# Autodesk Inventor assembly: axis3
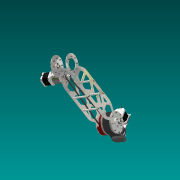
[picture p0: Inventor's stored thumbnail of the model, 180x180]
Saved by Autodesk Inventor 2020 (Build 240168000, 168)
## iProperties
Created: 2020-05-24
Part Number: axis3
Document SubType Name: Assembly
Designer: Svend
Author: Svend
## Documents named in this file (27)
- D:\github_gedeeld\BeerMinder\3D-model\axis3\axis3.iam
- D:\github_gedeeld\BeerMinder\3D-model\subAssembly\Nema17MetGearbox.iam
- D:\github_gedeeld\BeerMinder\3D-model\pulleys\GT2 Timing Pulley 20T - 8mm as.ipt
- D:\github_gedeeld\BeerMinder\3D-model\pulleys\Tandriem20naar60T-696mm.ipt
- D:\github_gedeeld\BeerMinder\3D-model\Base (Axis 1)\spiebaanBevestiging.ipt
- D:\github_gedeeld\BeerMinder\3D-model\pulleys\GT2 Timing Pulley 60T - 8mm as.ipt
- D:\github_gedeeld\BeerMinder\3D-model\bearings\Ball Bearing 608ZZ.ipt
- D:\github_gedeeld\BeerMinder\3D-model\Base (Axis 1)\asArm2.ipt
- D:\github_gedeeld\BeerMinder\3D-model\Base (Axis 1)\arm1v2.ipt
- D:\github_gedeeld\BeerMinder\3D-model\Base (Axis 1)\60mmspacer.ipt
- D:\github_gedeeld\BeerMinder\3D-model\Base (Axis 1)\60mmspacerDicht.ipt
- D:\github_gedeeld\BeerMinder\3D-model\bearings\stelring - 8mm.ipt
- D:\github_gedeeld\BeerMinder\3D-model\axis4\spacerVoorLager.ipt
- D:\github_gedeeld\BeerMinder\3D-model\boutjesEnMoertjes\ISO 4762 - M3 x 10ISO.ipt
- D:\github_gedeeld\BeerMinder\3D-model\boutjesEnMoertjes\ISO 7089 - 3 - 140 HV(1).ipt
- D:\github_gedeeld\BeerMinder\3D-model\boutjesEnMoertjes\ISO 10642 - M3x12.ipt
- D:\github_gedeeld\BeerMinder\3D-model\boutjesEnMoertjes\ISO 4035 - M3 - ISO.ipt
- D:\github_gedeeld\BeerMinder\3D-model\Base (Axis 1)\spiebaanplaatKlein.ipt
- D:\github_gedeeld\BeerMinder\3D-model\boutjesEnMoertjes\ISO 7380-1 - M4 x 16.ipt
- D:\github_gedeeld\BeerMinder\3D-model\Base (Axis 1)\arm1 tweede kant.ipt
- D:\github_gedeeld\BeerMinder\3D-model\axis4\axis4.iam
- D:\github_gedeeld\BeerMinder\3D-model\boutjesEnMoertjes\ISO 7380-1 - M3 x 8.ipt
- C:\Users\stefa\Documents\Inventor\Content Center Files\R2020\en-US\ISO 7089\ISO 7089 - 3 - 140 HV(1).ipt
- D:\github_gedeeld\BeerMinder\3D-model\axis3\asjes.ipt
- C:\Users\stefa\Documents\Inventor\Content Center Files\R2020\en-US\ISO 7089\ISO 7089 - 4 - 140 HV(1).ipt
- C:\Users\stefa\Documents\Inventor\Content Center Files\R2020\en-US\ISO 4762(2)\ISO 4762 - M4 x 12ISO.ipt
- D:\github_gedeeld\BeerMinder\3D-model\boutjesEnMoertjes\ISO 4762 - M3 x 30ISO.ipt
## Components (122 placed, 25 different names)
1. Nema17MetGearbox:1 [sub-assembly] — Mate:9, Mate:33, Mate:34, Mate:35, Mate:41
2. GT2 Timing Pulley 20T - 8mm as:1 — Mate:9, Mate:91, Mate:92
3. Tandriem20naar60T-696mm:1 — Mate:91, Mate:92
4. spiebaanBevestiging:1 — Flush:4
5. GT2 Timing Pulley 60T - 8mm as:1
6. Ball Bearing 608ZZ:1
7. asArm2:1 — Mate:89, Mate:94, Mate:98, Mate:100
8. arm1v2:1 — Mate:22, Mate:23, Mate:36, Mate:37, Mate:38, Mate:39, Mate:40, Mate:43, Mate:45, Mate:59, Insert:3, Insert:4, Insert:5, Insert:6, Insert:7, Insert:8, Insert:9, Insert:10, Mate:69, Mate:76, Insert:42, Insert:43, Insert:44, Insert:45, Insert:46, Insert:47, Insert:48, Insert:49, Mate:95, Mate:97, Mate:109, Mate:110, Insert:86, Insert:87, Insert:89, Insert:90, Insert:109, Insert:128, Mate:117, Mate:118, Mate:119
9. 60mmspacer:1
10. 60mmspacerDicht:1 — Mate:47, Mate:49, Mate:51, Mate:53, Mate:103, Mate:104
11. stelring - 8mm:1 — Mate:102
12. spacerVoorLager:1 — Mate:22, Mate:23, Mate:59, Mate:101
13. spiebaanplaatKlein:1 — Mate:69, Flush:4, Mate:70, Mate:71, Mate:72, Mate:73, Mate:74, Mate:75, Mate:76
14. 60mmspacerDicht:2 — Mate:85, Mate:86, Mate:88, Mate:90, Mate:100, Insert:72, Insert:73, Insert:74, Insert:75
15. 60mmspacer:2 — Mate:85, Mate:86, Mate:87, Mate:98, Mate:99
16. Ball Bearing 608ZZ:2 — Mate:87, Mate:88
17. stelring - 8mm:2 — Mate:89, Mate:90
18. arm1 tweede kant:1 — Mate:94, Mate:95, Mate:97, Mate:99, Insert:50, Insert:51, Insert:52, Insert:53, Insert:54, Insert:55, Insert:56, Insert:57, Insert:58, Insert:59, Insert:60, Insert:61, Insert:62, Insert:63, Insert:64, Insert:65, Mate:112, Insert:81, Insert:82, Insert:83, Insert:85, Insert:130
19. axis4:1 [sub-assembly] — Mate:101, Mate:102
20. asjes:1 — Mate:112, Mate:113
21. asjes:3 — Mate:115, Mate:117
22. asjes:4 — Mate:114, Mate:119
23. asjes:5 — Mate:116, Mate:118
24. ISO 4762 M3 x 10:12 — Insert:136
25. ISO 4762 M3 x 10:11 — Insert:135
26. ISO 4762 M3 x 10:10 — Insert:134
27. ISO 4762 M3 x 10:9 — Insert:133
28. ISO 4762 M3 x 10:8 — Insert:132
29. ISO 4762 M3 x 10:7 — Insert:131
30. ISO 4762 M3 x 10:6 — Insert:130
31. ISO 4762 M3 x 30:25 — Insert:129
32. ISO 4762 M3 x 30:24 — Insert:128
33. ISO 4762 M3 x 30:23 — Insert:127
34. ISO 4762 M3 x 30:5 — Insert:109
35. ISO 4762 M3 x 30:4 — Insert:108
36. ISO 4762 M3 x 30:3 — Insert:107
37. ISO 4762 M3 x 30:2 — Insert:106
38. ISO 4762 M3 x 30:1 — Insert:105
39. ISO 4762 M3 x 10:5 — Insert:104
40. ISO 7089 4:11 — Insert:90, Insert:99
41. ISO 7089 4:10 — Insert:89, Insert:101
42. ISO 7089 4:8 — Insert:87, Insert:100
43. ISO 7089 4:7 — Insert:86, Insert:98
44. ISO 7089 4:6 — Insert:85, Insert:95
45. ISO 7089 4:4 — Insert:83, Insert:93
46. ISO 7089 4:3 — Insert:82, Insert:94
47. ISO 7089 4:2 — Insert:81, Insert:96
48. ISO 4762 M4 x 12:10 — Insert:101
49. ISO 4762 M4 x 12:9 — Insert:100
50. ISO 4762 M4 x 12:8 — Insert:99
51. ISO 4762 M4 x 12:7 — Insert:98
52. ISO 4762 M4 x 12:5 — Insert:96, Mate:114
53. ISO 4762 M4 x 12:4 — Insert:95, Mate:115
54. ISO 4762 M4 x 12:3 — Insert:94, Mate:116
55. ISO 4762 M4 x 12:2 — Insert:93, Mate:113
56. ISO 4035 M3:8 — Insert:79, Mate:120
57. ISO 4035 M3:7 — Insert:78, Mate:123
58. ISO 4035 M3:6 — Insert:77, Mate:121
59. ISO 4035 M3:5 — Insert:76, Mate:122
60. ISO 10642 M3x12:10 — Mate:110
61. ISO 10642 M3x12:9 — Mate:109
62. ISO 10642 M3x12:8 — Mate:123
63. ISO 10642 M3x12:7 — Mate:121
64. ISO 10642 M3x12:6 — Mate:122
65. ISO 10642 M3x12:5 — Mate:120
66. ISO 7089 3:12 — Insert:75, Insert:77
67. ISO 7089 3:11 — Insert:74, Insert:78
68. ISO 7089 3:10 — Insert:73, Insert:76
69. ISO 7089 3:9 — Insert:72, Insert:79
70. ISO 7089 3:20 — Insert:65, Insert:136
71. ISO 7089 3:19 — Insert:64, Insert:134
72. ISO 7089 3:18 — Insert:63, Insert:132
73. ISO 7089 3:17 — Insert:62
74. ISO 7089 3:16 — Insert:61, Insert:131
75. ISO 7089 3:15 — Insert:60, Insert:133
76. ISO 7089 3:14 — Insert:59, Insert:135
77. ISO 7089 3:13 — Insert:58, Insert:104
78. ISO 7380-1 M3 x 8:24 — Insert:57
79. ISO 7380-1 M3 x 8:17 — Insert:56
80. ISO 7380-1 M3 x 8:18 — Insert:55
81. ISO 7380-1 M3 x 8:19 — Insert:54
82. ISO 7380-1 M3 x 8:20 — Insert:53
83. ISO 7380-1 M3 x 8:21 — Insert:52
84. ISO 7380-1 M3 x 8:22 — Insert:51
85. ISO 7380-1 M3 x 8:23 — Insert:50
86. ISO 7380-1 M3 x 8:9 — Insert:42
87. ISO 7380-1 M3 x 8:10 — Insert:43
88. ISO 7380-1 M3 x 8:11 — Insert:44
89. ISO 7380-1 M3 x 8:12 — Insert:45
90. ISO 7380-1 M3 x 8:13 — Insert:46
91. ISO 7380-1 M3 x 8:14 — Insert:47
92. ISO 7380-1 M3 x 8:15 — Insert:48
93. ISO 7380-1 M3 x 8:16 — Insert:49
94. ISO 7380-1 M4 x 16:1 — Mate:70, Mate:71
95. ISO 7380-1 M4 x 16:3 — Mate:72, Mate:73
96. ISO 7380-1 M4 x 16:2 — Mate:74, Mate:75
97. ISO 4762 M3 x 10:1 — Mate:29, Mate:30, Mate:34
98. ISO 4762 M3 x 10:2 — Mate:25, Mate:26, Mate:35
99. ISO 4762 M3 x 10:3 — Mate:27, Mate:28, Mate:41
100. ISO 4762 M3 x 10:4 — Mate:31, Mate:32, Mate:33
101. ISO 7089 3:1 — Mate:25, Mate:26, Mate:36
102. ISO 7089 3:2 — Mate:27, Mate:28, Mate:37, Mate:38
103. ISO 7089 3:3 — Mate:29, Mate:30, Mate:39
104. ISO 7089 3:4 — Mate:31, Mate:32, Mate:40
105. ISO 10642 M3x12:2 — Mate:43, Mate:46, Mate:54
106. ISO 10642 M3x12:4 — Mate:45, Mate:52, Mate:56
107. ISO 7089 3:5 — Mate:46, Mate:47, Mate:55
108. ISO 7089 3:6 — Mate:49, Insert:1
109. ISO 7089 3:7 — Mate:51, Insert:2
110. ISO 7089 3:8 — Mate:52, Mate:53, Mate:57
111. ISO 4035 M3:1 — Mate:54, Mate:55
112. ISO 4035 M3:2 — Mate:56, Mate:57
113. ISO 4035 M3:3 — Insert:1, Mate:104
114. ISO 4035 M3:4 — Insert:2, Mate:103
115. ISO 7089 3:27 — Insert:3
116. ISO 7089 3:28 — Insert:4, Insert:107
117. ISO 7089 3:29 — Insert:5, Insert:105
118. ISO 7089 3:30 — Insert:6
119. ISO 7089 3:31 — Insert:7, Insert:129
120. ISO 7089 3:32 — Insert:8, Insert:127
121. ISO 7089 3:33 — Insert:9, Insert:106
122. ISO 7089 3:34 — Insert:10, Insert:108
## Relationships (170: Mate 91, Insert 74, Flush 4, Angle 1)
- [Mate]: Tandriem20naar60T-696mm:1 ↔ GT2 Timing Pulley 60T - 8mm as:1
- [Mate] (0.5 mm): Tandriem20naar60T-696mm:1 ↔ GT2 Timing Pulley 60T - 8mm as:1
- [Mate]: GT2 Timing Pulley 60T - 8mm as:1 ↔ Ball Bearing 608ZZ:1
- [Mate]: GT2 Timing Pulley 60T - 8mm as:1 ↔ Ball Bearing 608ZZ:1
- [Mate]: Ball Bearing 608ZZ:1 ↔ asArm2:1
- [Mate]: spiebaanBevestiging:1 ↔ arm1v2:1
- [Flush]: spiebaanBevestiging:1 ↔ arm1v2:1
- [Mate]: Nema17MetGearbox:1 ↔ arm1v2:1
- [Angle] (180 deg): Nema17MetGearbox:1 ↔ arm1v2:1
- Mate:9: Nema17MetGearbox:1 ↔ GT2 Timing Pulley 20T - 8mm as:1
- [Mate]: Nema17MetGearbox:1 ↔ arm1v2:1
- [Mate]: arm1v2:1 ↔ 60mmspacer:1
- [Mate]: arm1v2:1 ↔ 60mmspacer:1
- [Mate]: arm1v2:1 ↔ 60mmspacer:1
- [Flush]: Ball Bearing 608ZZ:1 ↔ 60mmspacer:1
- [Mate]: 60mmspacer:1 ↔ 60mmspacerDicht:1
- [Mate]: 60mmspacer:1 ↔ 60mmspacerDicht:1
- [Mate]: 60mmspacer:1 ↔ 60mmspacerDicht:1
- [Mate]: asArm2:1 ↔ stelring - 8mm:1
- [Mate]: 60mmspacerDicht:1 ↔ stelring - 8mm:1
- [Flush]: asArm2:1 ↔ stelring - 8mm:1
- [Mate]: arm1v2:1 ↔ stelring - 8mm:1
- [Mate]: spiebaanBevestiging:1 ↔ arm1v2:1
- Mate:22: arm1v2:1 ↔ spacerVoorLager:1
- Mate:23: arm1v2:1 ↔ spacerVoorLager:1
- Mate:25: ISO 4762 M3 x 10:2 ↔ ISO 7089 3:1
- Mate:26: ISO 4762 M3 x 10:2 ↔ ISO 7089 3:1
- Mate:27: ISO 4762 M3 x 10:3 ↔ ISO 7089 3:2
- Mate:28: ISO 4762 M3 x 10:3 ↔ ISO 7089 3:2
- Mate:29: ISO 4762 M3 x 10:1 ↔ ISO 7089 3:3
- Mate:30: ISO 4762 M3 x 10:1 ↔ ISO 7089 3:3
- Mate:31: ISO 4762 M3 x 10:4 ↔ ISO 7089 3:4
- Mate:32: ISO 4762 M3 x 10:4 ↔ ISO 7089 3:4
- Mate:33: Nema17MetGearbox:1 ↔ ISO 4762 M3 x 10:4
- Mate:34: Nema17MetGearbox:1 ↔ ISO 4762 M3 x 10:1
- Mate:35: Nema17MetGearbox:1 ↔ ISO 4762 M3 x 10:2
- Mate:36: arm1v2:1 ↔ ISO 7089 3:1
- Mate:37: arm1v2:1 ↔ ISO 7089 3:2
- Mate:38: arm1v2:1 ↔ ISO 7089 3:2
- Mate:39: arm1v2:1 ↔ ISO 7089 3:3
- Mate:40: arm1v2:1 ↔ ISO 7089 3:4
- Mate:41: Nema17MetGearbox:1 ↔ ISO 4762 M3 x 10:3
- Mate:43: arm1v2:1 ↔ ISO 10642 M3x12:2
- Mate:45: arm1v2:1 ↔ ISO 10642 M3x12:4
- Mate:46: ISO 10642 M3x12:2 ↔ ISO 7089 3:5
- Mate:47: 60mmspacerDicht:1 ↔ ISO 7089 3:5
- Mate:49: 60mmspacerDicht:1 ↔ ISO 7089 3:6
- Mate:51: 60mmspacerDicht:1 ↔ ISO 7089 3:7
- Mate:52: ISO 10642 M3x12:4 ↔ ISO 7089 3:8
- Mate:53: 60mmspacerDicht:1 ↔ ISO 7089 3:8
- Mate:54: ISO 10642 M3x12:2 ↔ ISO 4035 M3:1
- Mate:55: ISO 7089 3:5 ↔ ISO 4035 M3:1
- Mate:56: ISO 10642 M3x12:4 ↔ ISO 4035 M3:2
- Mate:57: ISO 7089 3:8 ↔ ISO 4035 M3:2
- Insert:1: ISO 7089 3:6 ↔ ISO 4035 M3:3
- Insert:2: ISO 7089 3:7 ↔ ISO 4035 M3:4
- Mate:59: arm1v2:1 ↔ spacerVoorLager:1
- Insert:3: arm1v2:1 ↔ ISO 7089 3:27
- Insert:4: arm1v2:1 ↔ ISO 7089 3:28
- Insert:5: arm1v2:1 ↔ ISO 7089 3:29
- Insert:6: arm1v2:1 ↔ ISO 7089 3:30
- Insert:7: arm1v2:1 ↔ ISO 7089 3:31
- Insert:8: arm1v2:1 ↔ ISO 7089 3:32
- Insert:9: arm1v2:1 ↔ ISO 7089 3:33
- Insert:10: arm1v2:1 ↔ ISO 7089 3:34
- Mate:69: arm1v2:1 ↔ spiebaanplaatKlein:1
- Flush:4: spiebaanBevestiging:1 ↔ spiebaanplaatKlein:1
- Mate:70: spiebaanplaatKlein:1 ↔ ISO 7380-1 M4 x 16:1
- Mate:71: spiebaanplaatKlein:1 ↔ ISO 7380-1 M4 x 16:1
- Mate:72: spiebaanplaatKlein:1 ↔ ISO 7380-1 M4 x 16:3
- Mate:73: spiebaanplaatKlein:1 ↔ ISO 7380-1 M4 x 16:3
- Mate:74: spiebaanplaatKlein:1 ↔ ISO 7380-1 M4 x 16:2
- Mate:75: spiebaanplaatKlein:1 ↔ ISO 7380-1 M4 x 16:2
- Mate:76: arm1v2:1 ↔ spiebaanplaatKlein:1
- Insert:42: arm1v2:1 ↔ ISO 7380-1 M3 x 8:9
- Insert:43: arm1v2:1 ↔ ISO 7380-1 M3 x 8:10
- Insert:44: arm1v2:1 ↔ ISO 7380-1 M3 x 8:11
- Insert:45: arm1v2:1 ↔ ISO 7380-1 M3 x 8:12
- Insert:46: arm1v2:1 ↔ ISO 7380-1 M3 x 8:13
- Insert:47: arm1v2:1 ↔ ISO 7380-1 M3 x 8:14
- Insert:48: arm1v2:1 ↔ ISO 7380-1 M3 x 8:15
- Insert:49: arm1v2:1 ↔ ISO 7380-1 M3 x 8:16
- Mate:85: 60mmspacerDicht:2 ↔ 60mmspacer:2
- Mate:86: 60mmspacerDicht:2 ↔ 60mmspacer:2
- Mate:87: 60mmspacer:2 ↔ Ball Bearing 608ZZ:2
- Mate:88: 60mmspacerDicht:2 ↔ Ball Bearing 608ZZ:2
- Mate:89: asArm2:1 ↔ stelring - 8mm:2
- Mate:90: 60mmspacerDicht:2 ↔ stelring - 8mm:2
- Mate:91: GT2 Timing Pulley 20T - 8mm as:1 ↔ Tandriem20naar60T-696mm:1
- Mate:92 (0.5 mm): GT2 Timing Pulley 20T - 8mm as:1 ↔ Tandriem20naar60T-696mm:1
- Mate:94: asArm2:1 ↔ arm1 tweede kant:1
- Mate:95: arm1v2:1 ↔ arm1 tweede kant:1
- Mate:97 (60.6 mm): arm1v2:1 ↔ arm1 tweede kant:1
- Mate:98: asArm2:1 ↔ 60mmspacer:2
- Mate:99: 60mmspacer:2 ↔ arm1 tweede kant:1
- Mate:100: asArm2:1 ↔ 60mmspacerDicht:2
- Mate:101: spacerVoorLager:1 ↔ axis4:1
- Mate:102: stelring - 8mm:1 ↔ axis4:1
- Mate:103: 60mmspacerDicht:1 ↔ ISO 4035 M3:4
- Mate:104: 60mmspacerDicht:1 ↔ ISO 4035 M3:3
- Insert:50: arm1 tweede kant:1 ↔ ISO 7380-1 M3 x 8:23
- Insert:51: arm1 tweede kant:1 ↔ ISO 7380-1 M3 x 8:22
- Insert:52: arm1 tweede kant:1 ↔ ISO 7380-1 M3 x 8:21
- Insert:53: arm1 tweede kant:1 ↔ ISO 7380-1 M3 x 8:20
- Insert:54: arm1 tweede kant:1 ↔ ISO 7380-1 M3 x 8:19
- Insert:55: arm1 tweede kant:1 ↔ ISO 7380-1 M3 x 8:18
- Insert:56: arm1 tweede kant:1 ↔ ISO 7380-1 M3 x 8:17
- Insert:57: arm1 tweede kant:1 ↔ ISO 7380-1 M3 x 8:24
- Insert:58: arm1 tweede kant:1 ↔ ISO 7089 3:13
- Insert:59: arm1 tweede kant:1 ↔ ISO 7089 3:14
- Insert:60: arm1 tweede kant:1 ↔ ISO 7089 3:15
- Insert:61: arm1 tweede kant:1 ↔ ISO 7089 3:16
- Insert:62: arm1 tweede kant:1 ↔ ISO 7089 3:17
- Insert:63: arm1 tweede kant:1 ↔ ISO 7089 3:18
- Insert:64: arm1 tweede kant:1 ↔ ISO 7089 3:19
- Insert:65: arm1 tweede kant:1 ↔ ISO 7089 3:20
- Insert:72: 60mmspacerDicht:2 ↔ ISO 7089 3:9
- Insert:73: 60mmspacerDicht:2 ↔ ISO 7089 3:10
- Insert:74: 60mmspacerDicht:2 ↔ ISO 7089 3:11
- Insert:75: 60mmspacerDicht:2 ↔ ISO 7089 3:12
- Mate:109: arm1v2:1 ↔ ISO 10642 M3x12:9
- Mate:110: arm1v2:1 ↔ ISO 10642 M3x12:10
- Insert:76: ISO 4035 M3:5 ↔ ISO 7089 3:10
- Insert:77: ISO 4035 M3:6 ↔ ISO 7089 3:12
- Insert:78: ISO 4035 M3:7 ↔ ISO 7089 3:11
- Insert:79: ISO 4035 M3:8 ↔ ISO 7089 3:9
- Mate:112: arm1 tweede kant:1 ↔ asjes:1
- Insert:81: arm1 tweede kant:1 ↔ ISO 7089 4:2
- Insert:82: arm1 tweede kant:1 ↔ ISO 7089 4:3
- Insert:83: arm1 tweede kant:1 ↔ ISO 7089 4:4
- Insert:85: arm1 tweede kant:1 ↔ ISO 7089 4:6
- Insert:86: arm1v2:1 ↔ ISO 7089 4:7
- Insert:87: arm1v2:1 ↔ ISO 7089 4:8
- Insert:89: arm1v2:1 ↔ ISO 7089 4:10
- Insert:90: arm1v2:1 ↔ ISO 7089 4:11
- Insert:93: ISO 7089 4:4 ↔ ISO 4762 M4 x 12:2
- Insert:94: ISO 7089 4:3 ↔ ISO 4762 M4 x 12:3
- Insert:95: ISO 7089 4:6 ↔ ISO 4762 M4 x 12:4
- Insert:96: ISO 7089 4:2 ↔ ISO 4762 M4 x 12:5
- Insert:98: ISO 7089 4:7 ↔ ISO 4762 M4 x 12:7
- Insert:99: ISO 7089 4:11 ↔ ISO 4762 M4 x 12:8
- Insert:100: ISO 7089 4:8 ↔ ISO 4762 M4 x 12:9
- Insert:101: ISO 7089 4:10 ↔ ISO 4762 M4 x 12:10
- Insert:104: ISO 4762 M3 x 10:5 ↔ ISO 7089 3:13
- Insert:105: ISO 4762 M3 x 30:1 ↔ ISO 7089 3:29
- Insert:106: ISO 4762 M3 x 30:2 ↔ ISO 7089 3:33
- Insert:107: ISO 4762 M3 x 30:3 ↔ ISO 7089 3:28
- Insert:108: ISO 4762 M3 x 30:4 ↔ ISO 7089 3:34
- Insert:109: arm1v2:1 ↔ ISO 4762 M3 x 30:5
- Insert:127: ISO 4762 M3 x 30:23 ↔ ISO 7089 3:32
- Insert:128: arm1v2:1 ↔ ISO 4762 M3 x 30:24
- Insert:129: ISO 4762 M3 x 30:25 ↔ ISO 7089 3:31
- Mate:113: asjes:1 ↔ ISO 4762 M4 x 12:2
- Mate:114: asjes:4 ↔ ISO 4762 M4 x 12:5
- Mate:115: asjes:3 ↔ ISO 4762 M4 x 12:4
- Mate:116: asjes:5 ↔ ISO 4762 M4 x 12:3
- Mate:117: arm1v2:1 ↔ asjes:3
- Mate:118: arm1v2:1 ↔ asjes:5
- Mate:119: arm1v2:1 ↔ asjes:4
- Insert:130: arm1 tweede kant:1 ↔ ISO 4762 M3 x 10:6
- Insert:131: ISO 4762 M3 x 10:7 ↔ ISO 7089 3:16
- Insert:132: ISO 4762 M3 x 10:8 ↔ ISO 7089 3:18
- Insert:133: ISO 4762 M3 x 10:9 ↔ ISO 7089 3:15
- Insert:134: ISO 4762 M3 x 10:10 ↔ ISO 7089 3:19
- Insert:135: ISO 4762 M3 x 10:11 ↔ ISO 7089 3:14
- Insert:136: ISO 4762 M3 x 10:12 ↔ ISO 7089 3:20
- Mate:120: ISO 4035 M3:8 ↔ ISO 10642 M3x12:5
- Mate:121: ISO 4035 M3:6 ↔ ISO 10642 M3x12:7
- Mate:122: ISO 4035 M3:5 ↔ ISO 10642 M3x12:6
- Mate:123: ISO 4035 M3:7 ↔ ISO 10642 M3x12:8
